# Autodesk Inventor assembly: ElectronicsEnclosure
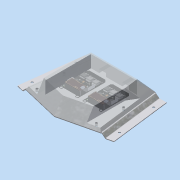
[picture p0: Inventor's stored thumbnail of the model, 180x180]
Saved by Autodesk Inventor 2015 (Build 190159000, 159)
## iProperties
Created: 2015-11-07
Part Number: ElectronicsEnclosure
Document SubType Name: Assembly
Designer: Raphael
Author: Raphael
## Documents named in this file (4)
- \\psf\Home\Documents\electric-skateboard\CAD\ElectronicsEnclosure.iam
- \\psf\Home\Documents\electric-skateboard\CAD\ElectronicsEnclosureBaseplate.ipt
- \\psf\Home\Documents\electric-skateboard\CAD\ElectronicsEnclosureCover.ipt
- \\psf\Home\Documents\electric-skateboard\CAD\ESC.ipt
## Components (4 placed, 3 different names)
1. ElectronicsEnclosureBaseplate:1 — Mate:1, Mate:2, Mate:3, Mate:4, Mate:5
2. ElectronicsEnclosureCover:1 — Mate:1, Mate:2, Mate:3
3. ESC:1 — Mate:5
4. ESC:2 — Mate:4
## Relationships (5: Mate 5)
- Mate:1: ElectronicsEnclosureBaseplate:1 ↔ ElectronicsEnclosureCover:1
- Mate:2: ElectronicsEnclosureBaseplate:1 ↔ ElectronicsEnclosureCover:1
- Mate:3: ElectronicsEnclosureBaseplate:1 ↔ ElectronicsEnclosureCover:1
- Mate:4: ElectronicsEnclosureBaseplate:1 ↔ ESC:2
- Mate:5: ElectronicsEnclosureBaseplate:1 ↔ ESC:1
